# Autodesk Inventor assembly: ODrive Pack
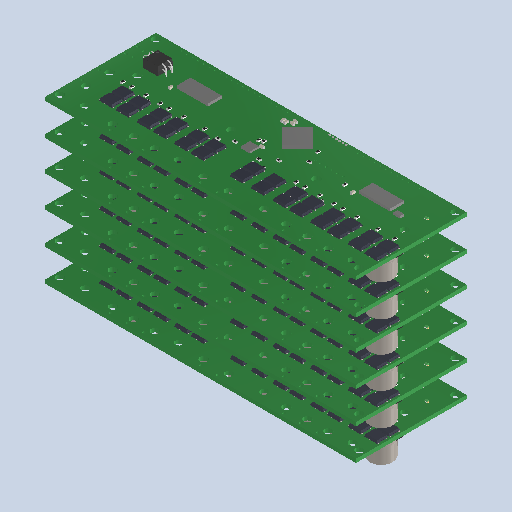
[picture p0: Inventor's stored thumbnail of the model, 512x512]
Saved by Autodesk Inventor 2023 (Build 270158000, 158)
## iProperties
Created: 2022-01-17
Part Number: ODrive Pack
Document SubType Name: Assembly
Designer: Jochen
Author: Jochen
## Documents named in this file (2)
- D:\Projects\Lisbeth\CAD\Common\odrive\ODrive Pack.iam
- D:\Projects\Lisbeth\CAD\Common\odrive\ODrive 3.5.iam
## Components (6 placed, 1 different names)
1. ODrive 3.5:1 [sub-assembly] — Angle:1, Flush:1, Flush:7, Flush:11
2. ODrive 3.5:2 [sub-assembly] — Angle:2, Flush:2, Flush:6, Flush:7, Flush:11, Flush:12
3. ODrive 3.5:3 [sub-assembly] — Angle:1, Angle:2, Flush:1, Flush:2, Flush:5, Flush:6, Flush:10, Flush:12, Flush:13
4. ODrive 3.5:4 [sub-assembly] — Flush:5, Flush:9, Flush:10, Flush:13, Flush:14
5. ODrive 3.5:5 [sub-assembly] — Flush:8, Flush:9, Flush:14, Flush:15
6. ODrive 3.5:6 [sub-assembly] — Flush:8, Flush:15
## Relationships (19: Flush 15, Angle 4)
- Angle:1 (0 deg): ODrive 3.5:1 ↔ ODrive 3.5:3
- Angle:2 (0 deg): ODrive 3.5:2 ↔ ODrive 3.5:3
- Flush:1: ODrive 3.5:1 ↔ ODrive 3.5:3
- Flush:2: ODrive 3.5:2 ↔ ODrive 3.5:3
- [Angle] (0 deg): ODrive 3.5:4 ↔ ODrive 3.5:6
- [Angle] (0 deg): ODrive 3.5:5 ↔ ODrive 3.5:6
- [Flush]: ODrive 3.5:4 ↔ ODrive 3.5:6
- [Flush]: ODrive 3.5:5 ↔ ODrive 3.5:6
- Flush:5: ODrive 3.5:3 ↔ ODrive 3.5:4
- Flush:6: ODrive 3.5:2 ↔ ODrive 3.5:3
- Flush:7: ODrive 3.5:1 ↔ ODrive 3.5:2
- Flush:8: ODrive 3.5:5 ↔ ODrive 3.5:6
- Flush:9: ODrive 3.5:4 ↔ ODrive 3.5:5
- Flush:10: ODrive 3.5:3 ↔ ODrive 3.5:4
- Flush:11: ODrive 3.5:1 ↔ ODrive 3.5:2
- Flush:12: ODrive 3.5:2 ↔ ODrive 3.5:3
- Flush:13: ODrive 3.5:3 ↔ ODrive 3.5:4
- Flush:14: ODrive 3.5:4 ↔ ODrive 3.5:5
- Flush:15: ODrive 3.5:5 ↔ ODrive 3.5:6
## Named parameters: d32_d28 = 0 deg, d33_d29 = 0 deg, d34_d30 = 0 mm, d35_d31 = 0 mm
